# Autodesk Inventor assembly: Optiweather caja
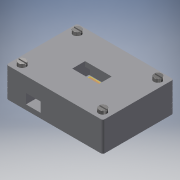
[picture p0: Inventor's stored thumbnail of the model, 180x180]
Saved by Autodesk Inventor 2017 (Build 210142000, 142)
## iProperties
Part Number: Optiweather caja
Material: Genérico
Document SubType Name: Assembly
Designer: user
Author: user
## Documents named in this file (8)
- C:\Users\user\Desktop\optiweather\Optiweather caja.iam
- C:\Users\user\Desktop\optiweather\placa electronica optiweather.ipt
- C:\Users\user\Desktop\optiweather\placa trasera.ipt
- C:\Users\user\Desktop\optiweather\Pieza3.ipt
- C:\Users\user\Desktop\optiweather\Pieza4.ipt
- C:\Users\user\Desktop\optiweather\Pieza5.ipt
- C:\Users\user\Desktop\optiweather\Pieza6.ipt
- C:\Users\user\Desktop\optiweather\Optiweather caja\Design Accelerator\Conexión por perno1.iam
## Components (8 placed, 7 different names)
1. placa electronica optiweather:1 — Coincidencia:1, Nivelación:1, Nivelación:2
2. placa trasera:1 — Coincidencia:1, Nivelación:1, Nivelación:2, Nivelación:3, Nivelación:4
3. Pieza3:1 — Nivelación:3, Nivelación:4, Coincidencia:2, Nivelación:5, Nivelación:6
4. Pieza3:2 — Coincidencia:2, Nivelación:5, Nivelación:6, Nivelación:7, Nivelación:8
5. Pieza4:1 — Nivelación:7, Nivelación:8, Nivelación:9, Nivelación:10
6. Pieza5:1 — Nivelación:9, Nivelación:10, Nivelación:11, Nivelación:12
7. Pieza6:1 — Nivelación:11, Nivelación:12, Coincidencia:3, Coincidencia:4
8. Conexión por perno:1 [sub-assembly] — Coincidencia:3, Coincidencia:4
## Relationships (16: Flush 12, Mate 4)
- Coincidencia:1 [Mate]: placa electronica optiweather:1 ↔ placa trasera:1
- Nivelación:1 [Flush] (-14 mm): placa electronica optiweather:1 ↔ placa trasera:1
- Nivelación:2 [Flush] (14 mm): placa electronica optiweather:1 ↔ placa trasera:1
- Nivelación:3 [Flush]: placa trasera:1 ↔ Pieza3:1
- Nivelación:4 [Flush]: placa trasera:1 ↔ Pieza3:1
- Coincidencia:2 [Mate]: Pieza3:1 ↔ Pieza3:2
- Nivelación:5 [Flush]: Pieza3:1 ↔ Pieza3:2
- Nivelación:6 [Flush]: Pieza3:1 ↔ Pieza3:2
- Nivelación:7 [Flush]: Pieza3:2 ↔ Pieza4:1
- Nivelación:8 [Flush]: Pieza3:2 ↔ Pieza4:1
- Nivelación:9 [Flush]: Pieza4:1 ↔ Pieza5:1
- Nivelación:10 [Flush]: Pieza4:1 ↔ Pieza5:1
- Nivelación:11 [Flush]: Pieza5:1 ↔ Pieza6:1
- Nivelación:12 [Flush]: Pieza5:1 ↔ Pieza6:1
- Coincidencia:3 [Mate]: Pieza6:1 ↔ Conexión por perno:1
- Coincidencia:4 [Mate]: Pieza6:1 ↔ Conexión por perno:1
